# Autodesk Inventor assembly: table
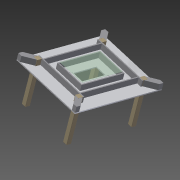
[picture p0: Inventor's stored thumbnail of the model, 180x180]
Saved by Autodesk Inventor 2015 (Build 190159000, 159)
## iProperties
Created: 2019-04-10
Part Number: table
Document SubType Name: Assembly
Designer: Raptor
Author: Raptor
## Documents named in this file (11)
- C:\Users\Raptor\Desktop\table\table.iam
- C:\Users\Raptor\Desktop\table\top long.ipt
- C:\Users\Raptor\Desktop\table\top short.ipt
- C:\Users\Raptor\Desktop\table\bottom long.ipt
- C:\Users\Raptor\Desktop\table\bottom short.ipt
- C:\Users\Raptor\Desktop\table\internal border long.ipt
- C:\Users\Raptor\Desktop\table\internal border short.ipt
- C:\Users\Raptor\Desktop\table\leg.ipt
- C:\Users\Raptor\Desktop\table\glass.ipt
- C:\Users\Raptor\Desktop\table\carrier plank long.ipt
- C:\Users\Raptor\Desktop\table\end.ipt
## Components (25 placed, 10 different names)
1. glass:1 — Mate:26, Mate:27, Flush:22
2. bottom long:1 — Mate:7, Mate:8, Flush:4, Mate:9, Flush:5, Mate:10, Mate:16
3. bottom short:1 — Mate:7, Mate:8, Flush:4, Mate:12
4. bottom short:2 — Mate:9, Flush:5, Mate:10, Mate:11, Flush:6, Flush:9, Mate:19
5. bottom long:2 — Mate:11, Flush:6, Mate:12, Flush:8, Mate:13, Mate:14
6. top short:2 — Mate:5, Flush:3, Mate:6, Flush:9, Flush:18, Mate:27, Flush:23, Flush:26, Mate:30, Flush:35, Flush:37
7. top long:2 — Mate:3, Flush:2, Mate:4, Mate:6, Flush:17, Mate:17, Mate:21, Mate:22, Mate:23, Mate:24, Flush:25, Flush:28, Mate:34, Mate:37, Flush:38, Mate:38, Flush:40
8. top short:1 — Mate:1, Mate:2, Flush:1, Mate:3, Flush:2, Mate:4, Mate:20, Flush:20, Flush:27, Flush:30, Mate:28, Flush:39, Mate:39, Flush:42
9. top long:1 — Mate:1, Mate:2, Flush:1, Mate:5, Flush:3, Flush:8, Mate:13, Flush:16, Mate:15, Mate:26, Flush:22, Flush:24, Flush:29, Mate:32, Mate:36, Flush:36, Flush:41
10. leg:1 — Mate:21, Flush:25, Flush:26
11. leg:2 — Mate:22, Flush:27, Flush:28
12. leg:3 — Mate:23, Flush:29, Flush:30, Mate:29, Flush:31
13. leg:4 — Mate:24, Flush:23, Flush:24, Mate:31, Flush:32
14. internal border long:1 — Mate:14, Flush:16, Mate:15
15. internal border long:2 — Mate:16, Flush:17, Mate:17, Flush:19, Flush:21
16. internal border short:1 — Mate:19, Flush:18, Flush:19
17. internal border short:2 — Mate:20, Flush:20, Flush:21
18. carrier plank long:1 — Mate:28, Mate:29, Flush:31
19. carrier plank long:2 — Mate:30, Mate:31, Flush:32, Mate:33, Flush:33, Mate:35, Flush:34
20. carrier plank long:3 — Mate:34, Mate:35, Flush:34
21. carrier plank long:4 — Mate:32, Mate:33, Flush:33
22. end:1 — Mate:36, Flush:35, Flush:36
23. end:2 — Mate:39, Flush:41, Flush:42
24. end:3 — Mate:38, Flush:39, Flush:40
25. end:4 — Mate:37, Flush:37, Flush:38
## Relationships (72: Mate 37, Flush 35)
- Mate:1: top short:1 ↔ top long:1
- Mate:2: top short:1 ↔ top long:1
- Flush:1: top short:1 ↔ top long:1
- Mate:3: top long:2 ↔ top short:1
- Flush:2: top long:2 ↔ top short:1
- Mate:4: top long:2 ↔ top short:1
- Mate:5: top short:2 ↔ top long:1
- Flush:3: top short:2 ↔ top long:1
- Mate:6: top short:2 ↔ top long:2
- Mate:7: bottom long:1 ↔ bottom short:1
- Mate:8: bottom long:1 ↔ bottom short:1
- Flush:4: bottom long:1 ↔ bottom short:1
- Mate:9: bottom long:1 ↔ bottom short:2
- Flush:5: bottom long:1 ↔ bottom short:2
- Mate:10: bottom long:1 ↔ bottom short:2
- Mate:11: bottom short:2 ↔ bottom long:2
- Flush:6: bottom short:2 ↔ bottom long:2
- Mate:12: bottom short:1 ↔ bottom long:2
- Flush:8: bottom long:2 ↔ top long:1
- Flush:9: bottom short:2 ↔ top short:2
- Mate:13 (100 mm): bottom long:2 ↔ top long:1
- Mate:14: bottom long:2 ↔ internal border long:1
- Flush:16: top long:1 ↔ internal border long:1
- Mate:15: top long:1 ↔ internal border long:1
- Mate:16: bottom long:1 ↔ internal border long:2
- Flush:17: top long:2 ↔ internal border long:2
- Mate:17: top long:2 ↔ internal border long:2
- Mate:19: bottom short:2 ↔ internal border short:1
- Flush:18: top short:2 ↔ internal border short:1
- Flush:19: internal border long:2 ↔ internal border short:1
- Mate:20: top short:1 ↔ internal border short:2
- Flush:20: top short:1 ↔ internal border short:2
- Flush:21: internal border long:2 ↔ internal border short:2
- Mate:21: top long:2 ↔ leg:1
- Mate:22: top long:2 ↔ leg:2
- Mate:23: top long:2 ↔ leg:3
- Mate:24: top long:2 ↔ leg:4
- Mate:26: glass:1 ↔ top long:1
- Mate:27: glass:1 ↔ top short:2
- Flush:22: glass:1 ↔ top long:1
- Flush:23 (150 mm): top short:2 ↔ leg:4
- Flush:24 (150 mm): top long:1 ↔ leg:4
- Flush:25 (-150 mm): top long:2 ↔ leg:1
- Flush:26 (-150 mm): top short:2 ↔ leg:1
- Flush:27 (150 mm): top short:1 ↔ leg:2
- Flush:28 (150 mm): top long:2 ↔ leg:2
- Flush:29 (150 mm): top long:1 ↔ leg:3
- Flush:30 (-150 mm): top short:1 ↔ leg:3
- Mate:28: top short:1 ↔ carrier plank long:1
- Mate:29: leg:3 ↔ carrier plank long:1
- Flush:31: leg:3 ↔ carrier plank long:1
- Mate:30: top short:2 ↔ carrier plank long:2
- Mate:31: leg:4 ↔ carrier plank long:2
- Flush:32: leg:4 ↔ carrier plank long:2
- Mate:32: top long:1 ↔ carrier plank long:4
- Mate:33: carrier plank long:2 ↔ carrier plank long:4
- Flush:33 (80 mm): carrier plank long:2 ↔ carrier plank long:4
- Mate:34: top long:2 ↔ carrier plank long:3
- Mate:35: carrier plank long:2 ↔ carrier plank long:3
- Flush:34 (80 mm): carrier plank long:2 ↔ carrier plank long:3
- Mate:36: top long:1 ↔ end:1
- Flush:35: top short:2 ↔ end:1
- Flush:36: top long:1 ↔ end:1
- Mate:37: top long:2 ↔ end:4
- Flush:37: top short:2 ↔ end:4
- Flush:38: top long:2 ↔ end:4
- Mate:38: top long:2 ↔ end:3
- Flush:39: top short:1 ↔ end:3
- Flush:40: top long:2 ↔ end:3
- Mate:39: top short:1 ↔ end:2
- Flush:41: top long:1 ↔ end:2
- Flush:42: top short:1 ↔ end:2
